# Autodesk Inventor assembly: back shell
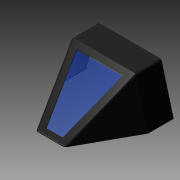
[picture p0: Inventor's stored thumbnail of the model, 180x180]
Saved by Autodesk Inventor 2012 (Build 160160000, 160)
## iProperties
Created: 2011-12-02
Part Number: back shell
Document SubType Name: Assembly
Designer: Antonella
Author: Antonella
## Documents named in this file (3)
- C:\Users\Antonella\Documents\GCC Robotics 2012 - Mechanical\Robot 2.0\Weatherproofing Shell\back shell.iam
- C:\Users\Antonella\Documents\GCC Robotics 2012 - Mechanical\Robot 2.0\Weatherproofing Shell\back shell.ipt
- C:\Users\Antonella\Documents\GCC Robotics 2012 - Mechanical\Robot 2.0\Weatherproofing Shell\back window.ipt
## Components (2 placed, 2 different names)
1. back shell:1 — Mate:1, Mate:2
2. back window:1 — Mate:1, Mate:2, Mate:3
## Relationships (3: Mate 3)
- Mate:1: back shell:1 ↔ back window:1
- Mate:2 (6.35 mm): back shell:1 ↔ back window:1
- Mate:3: back window:1
